# Autodesk Inventor assembly: 19th_jianjeong_04
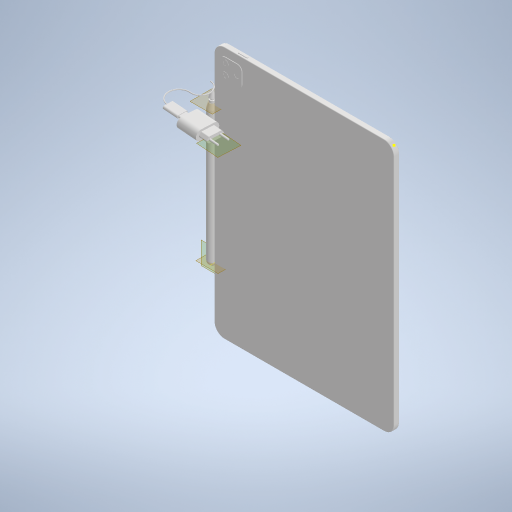
[picture p0: Inventor's stored thumbnail of the model, 512x512]
Saved by Autodesk Inventor 2024.3 (Build 283343000, 343)
## iProperties
Created: 2024-08-06
Part Number: 19th_jianjeong_04
Document SubType Name: Assembly
Designer: naru4
Author: naru4
## Documents named in this file (6)
- C:\Users\naru4\OneDrive\바탕 화면\19th_jianjeong_04.iam
- C:\Users\naru4\OneDrive\바탕 화면\apple pensil tip.ipt
- C:\Users\naru4\OneDrive\바탕 화면\apple pensil.ipt
- C:\Users\naru4\OneDrive\바탕 화면\Ctype addapter.ipt
- C:\Users\naru4\OneDrive\바탕 화면\ctype charger.ipt
- C:\Users\naru4\OneDrive\바탕 화면\ipad.ipt
## Components (5 placed, 5 different names)
1. apple pensil tip:1 — 회전:1
2. apple pensil:1 — 회전:1, 강체:1
3. Ctype addapter:1 — 회전:2
4. ctype charger:1 — 회전:2
5. ipad:1 — 강체:1
## Relationships (3: RevoluteJoint 2, WeldJoint 1)
- 회전:1 [RevoluteJoint]: apple pensil tip:1 ↔ apple pensil:1
- 회전:2 [RevoluteJoint]: Ctype addapter:1 ↔ ctype charger:1
- 강체:1 [WeldJoint]: apple pensil:1 ↔ ipad:1
